# Autodesk Inventor assembly: grabber assembly
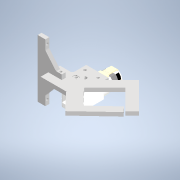
[picture p0: Inventor's stored thumbnail of the model, 180x180]
Saved by Autodesk Inventor 2020.1 (Build 241239000, 239)
## iProperties
Created: 2019-10-24
Part Number: grabber assembly
Document SubType Name: Assembly
Designer: amirs
Author: amirs
## Documents named in this file (6)
- C:\Users\amirs\Downloads\grabber assembly.iam
- C:\Users\amirs\Downloads\axle extender.ipt
- C:\Users\amirs\Downloads\Solarbotics_GM9-Assem.iam
- C:\Users\amirs\Downloads\gripper (moving part.ipt
- C:\Users\amirs\Downloads\gripper laser cut.ipt
- C:\Users\amirs\Downloads\mount laser cut.ipt
## Components (5 placed, 5 different names)
1. axle extender:1 — Mate:4, Mate:5, Mate:6, Mate:7
2. Solarbotics_GM9-Assem:1 [sub-assembly] — Mate:4, Mate:5, Mate:8, Mate:9, Mate:10, Mate:15
3. gripper (moving part:1 — Mate:6, Mate:7
4. gripper laser cut:1 — Mate:8, Mate:9, Mate:10, Mate:12, Mate:13, Mate:14
5. mount laser cut:1 — Mate:12, Mate:13, Mate:14
## Relationships (11: Mate 11)
- Mate:4: axle extender:1 ↔ Solarbotics_GM9-Assem:1
- Mate:5: axle extender:1 ↔ Solarbotics_GM9-Assem:1
- Mate:6: axle extender:1 ↔ gripper (moving part:1
- Mate:7: axle extender:1 ↔ gripper (moving part:1
- Mate:8: Solarbotics_GM9-Assem:1 ↔ gripper laser cut:1
- Mate:9: Solarbotics_GM9-Assem:1 ↔ gripper laser cut:1
- Mate:10: Solarbotics_GM9-Assem:1 ↔ gripper laser cut:1
- Mate:12: gripper laser cut:1 ↔ mount laser cut:1
- Mate:13: gripper laser cut:1 ↔ mount laser cut:1
- Mate:14: gripper laser cut:1 ↔ mount laser cut:1
- Mate:15: Solarbotics_GM9-Assem:1
